# Autodesk Inventor assembly: tsop
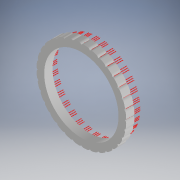
[picture p0: Inventor's stored thumbnail of the model, 180x180]
Saved by Autodesk Inventor 2020 (Build 240168000, 168)
## iProperties
Created: 2024-11-04
Part Number: tsop
Document SubType Name: Assembly
Designer: Ivan
Author: Ivan
## Documents named in this file (3)
- C:\!projects\DASH_\3D\Dash-V1\tsop.iam
- C:\!projects\DASH_\3D\Dash-V1\tsop_lid.ipt
- C:\!projects\DASH_\3D\Dash-V1\step\tssp58038.ipt
## Components (33 placed, 2 different names)
1. tsop_lid:1 — Совмещение:1, Заподлицо:1, Угол:1, Угол:2, Угол:3, Совмещение:2, Совмещение:3, Совмещение:4
2. tssp58038:1 — Угол:1, Угол:3, Совмещение:2, Совмещение:3, Совмещение:4
3. tssp58038:2
4. tssp58038:3
5. tssp58038:4
6. tssp58038:5
7. tssp58038:6
8. tssp58038:7
9. tssp58038:8
10. tssp58038:9
11. tssp58038:10
12. tssp58038:11
13. tssp58038:12
14. tssp58038:13
15. tssp58038:14
16. tssp58038:15
17. tssp58038:16
18. tssp58038:17
19. tssp58038:18
20. tssp58038:19
21. tssp58038:20
22. tssp58038:21
23. tssp58038:22
24. tssp58038:23
25. tssp58038:24
26. tssp58038:25
27. tssp58038:26
28. tssp58038:27
29. tssp58038:28
30. tssp58038:29
31. tssp58038:30
32. tssp58038:31
33. tssp58038:32
## Component patterns: (32 elements, first: tssp58038:1)
## Relationships (8: Mate 4, Angle 3, Flush 1)
- Совмещение:1 [Mate]: tsop_lid:1
- Заподлицо:1 [Flush]: tsop_lid:1
- Угол:1 [Angle] (0 deg): tsop_lid:1 ↔ tssp58038:1
- Угол:2 [Angle] (0 deg): tsop_lid:1
- Угол:3 [Angle] (0 deg): tsop_lid:1 ↔ tssp58038:1
- Совмещение:2 [Mate]: tsop_lid:1 ↔ tssp58038:1
- Совмещение:3 [Mate]: tsop_lid:1 ↔ tssp58038:1
- Совмещение:4 [Mate]: tsop_lid:1 ↔ tssp58038:1
